# Autodesk Inventor assembly: robotis_pi_box
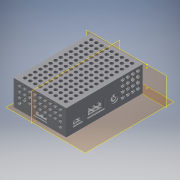
[picture p0: Inventor's stored thumbnail of the model, 180x180]
Saved by Autodesk Inventor 2016 (Build 200138000, 138)
## iProperties
Created: 2016-02-13
Part Number: robotis_pi_box
Document SubType Name: Assembly
Designer: jforce
Author: jforce
## Documents named in this file (3)
- C:\Users\jforce\Dropbox\gmu\ece590\robot_models\robotis_pi_box.iam
- C:\Users\jforce\Dropbox\gmu\ece590\robot_models\rpi2-top3.ipt
- C:\Users\jforce\Dropbox\gmu\ece590\robot_models\rpi2-bottom4.ipt
## Components (2 placed, 2 different names)
1. rpi2-top3:1 — Flush:1, Mate:4, Flush:2
2. rpi2-bottom4:1 — Mate:1, Mate:2, Mate:3, Flush:1, Mate:4, Flush:2
## Relationships (6: Mate 4, Flush 2)
- Mate:1: rpi2-bottom4:1
- Mate:2 (-25.4 mm): rpi2-bottom4:1
- Mate:3: rpi2-bottom4:1
- Flush:1: rpi2-top3:1 ↔ rpi2-bottom4:1
- Mate:4: rpi2-top3:1 ↔ rpi2-bottom4:1
- Flush:2: rpi2-top3:1 ↔ rpi2-bottom4:1
